# Autodesk Inventor assembly: Anglerfish_bonne_mamman_m12large_flipped_v0
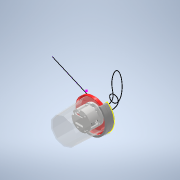
[picture p0: Inventor's stored thumbnail of the model, 180x180]
Saved by Autodesk Inventor 2022 (Build 260153000, 153)
## iProperties
Created: 2022-04-02
Part Number: Anglerfish_bonne_mamman_m12large_flipped_v0
Document SubType Name: Assembly
Designer: Prakash Lab
Author: Prakash Lab
## Documents named in this file (18)
- C:\Users\diederichbenedict\Dropbox\Dokumente\Promotion\PROJECTS\Matchboxscope\INVENTOR\ANGLERFISH\Anglerfish_bonne_mamman_m12large_flipped_v0.iam
- C:\Users\diederichbenedict\Dropbox\Dokumente\Promotion\PROJECTS\Matchboxscope\INVENTOR\ANGLERFISH\00_ESP3-CAM.iam
- C:\Users\diederichbenedict\Dropbox\Dokumente\Promotion\PROJECTS\Matchboxscope\INVENTOR\ANGLERFISH\00_Powerbank.ipt
- C:\Users\diederichbenedict\Dropbox\Dokumente\Promotion\PROJECTS\Matchboxscope\INVENTOR\ANGLERFISH\00_bonne_maman_jar.ipt
- C:\Users\diederichbenedict\Dropbox\Dokumente\Promotion\PROJECTS\Matchboxscope\INVENTOR\ANGLERFISH\Matchboxscope_M12_Lensadapter_v0.ipt
- C:\Users\diederichbenedict\Dropbox\Dokumente\Promotion\PROJECTS\Matchboxscope\INVENTOR\ANGLERFISH\00_toslink_launcher_v3.ipt
- C:\Users\diederichbenedict\Dropbox\Dokumente\Promotion\PROJECTS\Matchboxscope\INVENTOR\ANGLERFISH\00_CCTV_M12_VCM_large.ipt
- C:\Users\diederichbenedict\Dropbox\Dokumente\Promotion\PROJECTS\Matchboxscope\INVENTOR\ANGLERFISH\Anglerfish_flipped_LidMoun.ipt
- C:\Users\diederichbenedict\Dropbox\Dokumente\Promotion\PROJECTS\Matchboxscope\INVENTOR\ANGLERFISH\Anglerfish_flipped_Baselayer.ipt
- C:\Users\diederichbenedict\Dropbox\Dokumente\Promotion\PROJECTS\Matchboxscope\INVENTOR\ANGLERFISH\Anglerfish_flipped_Electronicsmount.ipt
- C:\Users\diederichbenedict\Dropbox\Dokumente\Promotion\PROJECTS\Matchboxscope\INVENTOR\ANGLERFISH\00_Coverglass.ipt
- C:\Users\diederichbenedict\Dropbox\Dokumente\Promotion\PROJECTS\Matchboxscope\INVENTOR\ANGLERFISH\00_Lid_Bonne_Mamman.ipt
- C:\Users\diederichbenedict\Dropbox\Dokumente\Promotion\PROJECTS\Matchboxscope\INVENTOR\ANGLERFISH\00_Magnet_8x3mm.ipt
- C:\Users\UC2\Documents\Inventor\Content Center Files\R2022\de-DE\DIN 912\DIN 912 - M3 x 0,5 x 12 x 10,75.ipt
- C:\Users\diederichbenedict\Dropbox\Dokumente\Promotion\PROJECTS\Matchboxscope\INVENTOR\ANGLERFISH\00_Toslink.ipt
- C:\Users\diederichbenedict\Dropbox\Dokumente\Promotion\PROJECTS\Matchboxscope\INVENTOR\ANGLERFISH\Anglerfish_Lightplate_Tosslink_adjuster_flipped.ipt
- C:\Users\diederichbenedict\Documents\Inventor\Content Center Files\R2022\de-DE\DIN 912\DIN 912 - M3 x 0.5 x 8 x 6.75.ipt
- C:\Users\diederichbenedict\Dropbox\Dokumente\Promotion\PROJECTS\Matchboxscope\INVENTOR\ANGLERFISH\Anglerfish_Lightplate_Tosslink_base_flipped.ipt
## Components (33 placed, 17 different names)
1. 00_Powerbank:1
2. 00_bonne_maman_jar:1 — Passend:10, Winkel:1, Fluchtend:1
3. 00_ESP3-CAM:1 [sub-assembly] — Passend:23, Passend:24, Winkel:9, Winkel:11
4. 00_CCTV_M12_VCM_large:1 — Passend:30, Fluchtend:3, Einfügen:11
5. Matchboxscope_M12_Lensadapter_v0:1 — Einfügen:11
6. Anglerfish_flipped_Electronicsmount:1 — Einfügen:2, Winkel:11, Passend:30
7. Anglerfish_flipped_LidMoun:1 — Einfügen:3, Einfügen:5, Einfügen:6, Einfügen:7
8. Anglerfish_flipped_Baselayer:1 — Passend:23, Passend:24, Winkel:9, Einfügen:2, Winkel:10, Fluchtend:3, Einfügen:8, Einfügen:9, Einfügen:10, Einfügen:12, Einfügen:13, Einfügen:14, Einfügen:15, Einfügen:16, Einfügen:17
9. 00_Coverglass:1 — Passend:25, Passend:26, Fluchtend:2
10. 00_Lid_Bonne_Mamman:1 — Einfügen:3, Winkel:12, Passend:25, Passend:26, Passend:27
11. Anglerfish_Lightplate_Tosslink_base_flipped:1 — Passend:27, Fluchtend:2, Fluchtend:4, Fluchtend:5, Einfügen:20, Einfügen:21, Einfügen:22, Einfügen:23, Einfügen:24, Einfügen:25
12. 00_Magnet_8x3mm:1 — Einfügen:7
13. 00_Magnet_8x3mm:2 — Einfügen:5
14. 00_Magnet_8x3mm:3 — Einfügen:9
15. 00_Magnet_8x3mm:4 — Einfügen:6
16. 00_Magnet_8x3mm:5 — Einfügen:8
17. 00_Magnet_8x3mm:6 — Einfügen:10
18. DIN 912 - ersetzt durch DIN EN ISO 4762 M3 x 12:1 — Einfügen:14
19. DIN 912 - ersetzt durch DIN EN ISO 4762 M3 x 12:2 — Einfügen:17
20. DIN 912 - ersetzt durch DIN EN ISO 4762 M3 x 12:4 — Einfügen:15
21. DIN 912 - ersetzt durch DIN EN ISO 4762 M3 x 12:5 — Einfügen:12
22. DIN 912 - ersetzt durch DIN EN ISO 4762 M3 x 12:6 — Einfügen:16
23. DIN 912 - ersetzt durch DIN EN ISO 4762 M3 x 12:7 — Einfügen:13
24. 00_Toslink:1
25. Anglerfish_Lightplate_Tosslink_adjuster_flipped:1 — Fluchtend:4, Fluchtend:5, Einfügen:18, Einfügen:19
26. 00_toslink_launcher_v3:3 — Einfügen:19
27. 00_toslink_launcher_v3:4 — Einfügen:18
28. DIN 912 - ersetzt durch DIN EN ISO 4762 M3 x 8:1 — Einfügen:23
29. DIN 912 - ersetzt durch DIN EN ISO 4762 M3 x 8:2 — Einfügen:21
30. DIN 912 - ersetzt durch DIN EN ISO 4762 M3 x 8:3 — Einfügen:22
31. DIN 912 - ersetzt durch DIN EN ISO 4762 M3 x 8:4 — Einfügen:24
32. DIN 912 - ersetzt durch DIN EN ISO 4762 M3 x 8:5 — Einfügen:20
33. DIN 912 - ersetzt durch DIN EN ISO 4762 M3 x 8:6 — Einfügen:25
## Relationships (41: Insert 23, Mate 7, Angle 6, Flush 5)
- Passend:10 [Mate]: 00_bonne_maman_jar:1
- Winkel:1 [Angle] (0 deg): 00_bonne_maman_jar:1
- Fluchtend:1 [Flush]: 00_bonne_maman_jar:1
- [Angle] (45 deg): Anglerfish_flipped_Electronicsmount:1 ↔ Anglerfish_flipped_LidMoun:1
- Passend:23 [Mate]: 00_ESP3-CAM:1 ↔ Anglerfish_flipped_Baselayer:1
- Passend:24 [Mate]: 00_ESP3-CAM:1 ↔ Anglerfish_flipped_Baselayer:1
- Winkel:9 [Angle] (180 deg): 00_ESP3-CAM:1 ↔ Anglerfish_flipped_Baselayer:1
- Einfügen:2 [Insert]: Anglerfish_flipped_Electronicsmount:1 ↔ Anglerfish_flipped_Baselayer:1
- Winkel:10 [Angle] (180 deg): Anglerfish_flipped_Baselayer:1
- Winkel:11 [Angle] (180 deg): 00_ESP3-CAM:1 ↔ Anglerfish_flipped_Electronicsmount:1
- Einfügen:3 [Insert]: Anglerfish_flipped_LidMoun:1 ↔ 00_Lid_Bonne_Mamman:1
- Winkel:12 [Angle] (0 deg): 00_Lid_Bonne_Mamman:1
- Passend:25 [Mate]: 00_Coverglass:1 ↔ 00_Lid_Bonne_Mamman:1
- Passend:26 [Mate]: 00_Coverglass:1 ↔ 00_Lid_Bonne_Mamman:1
- Passend:27 [Mate]: 00_Lid_Bonne_Mamman:1 ↔ Anglerfish_Lightplate_Tosslink_base_flipped:1
- Fluchtend:2 [Flush]: 00_Coverglass:1 ↔ Anglerfish_Lightplate_Tosslink_base_flipped:1
- Passend:30 [Mate]: 00_CCTV_M12_VCM_large:1 ↔ Anglerfish_flipped_Electronicsmount:1
- Fluchtend:3 [Flush]: 00_CCTV_M12_VCM_large:1 ↔ Anglerfish_flipped_Baselayer:1
- Einfügen:5 [Insert]: Anglerfish_flipped_LidMoun:1 ↔ 00_Magnet_8x3mm:2
- Einfügen:6 [Insert]: Anglerfish_flipped_LidMoun:1 ↔ 00_Magnet_8x3mm:4
- Einfügen:7 [Insert]: Anglerfish_flipped_LidMoun:1 ↔ 00_Magnet_8x3mm:1
- Einfügen:8 [Insert]: Anglerfish_flipped_Baselayer:1 ↔ 00_Magnet_8x3mm:5
- Einfügen:9 [Insert]: Anglerfish_flipped_Baselayer:1 ↔ 00_Magnet_8x3mm:3
- Einfügen:10 [Insert]: Anglerfish_flipped_Baselayer:1 ↔ 00_Magnet_8x3mm:6
- Einfügen:11 [Insert]: 00_CCTV_M12_VCM_large:1 ↔ Matchboxscope_M12_Lensadapter_v0:1
- Einfügen:12 [Insert]: Anglerfish_flipped_Baselayer:1 ↔ DIN 912 - ersetzt durch DIN EN ISO 4762 M3 x 12:5
- Einfügen:13 [Insert]: Anglerfish_flipped_Baselayer:1 ↔ DIN 912 - ersetzt durch DIN EN ISO 4762 M3 x 12:7
- Einfügen:14 [Insert]: Anglerfish_flipped_Baselayer:1 ↔ DIN 912 - ersetzt durch DIN EN ISO 4762 M3 x 12:1
- Einfügen:15 [Insert]: Anglerfish_flipped_Baselayer:1 ↔ DIN 912 - ersetzt durch DIN EN ISO 4762 M3 x 12:4
- Einfügen:16 [Insert]: Anglerfish_flipped_Baselayer:1 ↔ DIN 912 - ersetzt durch DIN EN ISO 4762 M3 x 12:6
- Einfügen:17 [Insert]: Anglerfish_flipped_Baselayer:1 ↔ DIN 912 - ersetzt durch DIN EN ISO 4762 M3 x 12:2
- Fluchtend:4 [Flush]: Anglerfish_Lightplate_Tosslink_base_flipped:1 ↔ Anglerfish_Lightplate_Tosslink_adjuster_flipped:1
- Fluchtend:5 [Flush]: Anglerfish_Lightplate_Tosslink_base_flipped:1 ↔ Anglerfish_Lightplate_Tosslink_adjuster_flipped:1
- Einfügen:18 [Insert]: Anglerfish_Lightplate_Tosslink_adjuster_flipped:1 ↔ 00_toslink_launcher_v3:4
- Einfügen:19 [Insert]: Anglerfish_Lightplate_Tosslink_adjuster_flipped:1 ↔ 00_toslink_launcher_v3:3
- Einfügen:20 [Insert] (2 mm): Anglerfish_Lightplate_Tosslink_base_flipped:1 ↔ DIN 912 - ersetzt durch DIN EN ISO 4762 M3 x 8:5
- Einfügen:21 [Insert] (2 mm): Anglerfish_Lightplate_Tosslink_base_flipped:1 ↔ DIN 912 - ersetzt durch DIN EN ISO 4762 M3 x 8:2
- Einfügen:22 [Insert] (2 mm): Anglerfish_Lightplate_Tosslink_base_flipped:1 ↔ DIN 912 - ersetzt durch DIN EN ISO 4762 M3 x 8:3
- Einfügen:23 [Insert] (2 mm): Anglerfish_Lightplate_Tosslink_base_flipped:1 ↔ DIN 912 - ersetzt durch DIN EN ISO 4762 M3 x 8:1
- Einfügen:24 [Insert] (2 mm): Anglerfish_Lightplate_Tosslink_base_flipped:1 ↔ DIN 912 - ersetzt durch DIN EN ISO 4762 M3 x 8:4
- Einfügen:25 [Insert] (2 mm): Anglerfish_Lightplate_Tosslink_base_flipped:1 ↔ DIN 912 - ersetzt durch DIN EN ISO 4762 M3 x 8:6
